# Autodesk Inventor assembly: 3D Printed PCR
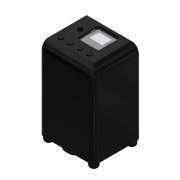
[picture p0: Inventor's stored thumbnail of the model, 180x180]
Saved by Autodesk Inventor 2017 (Build 210142000, 142)
## iProperties
Created: 2017-01-30
Part Number: 3D Printed PCR
Document SubType Name: Assembly
Designer: ge937963
Author: ge937963
## Documents named in this file (8)
- C:\Users\ge937963\Desktop\Inventor View\3D Printed PCR.iam
- C:\Users\ge937963\Desktop\Inventor View\Control Assembly.iam
- C:\Users\ge937963\Desktop\Inventor View\Case.ipt
- C:\Users\ge937963\Desktop\Inventor View\Photodiode Assembly.iam
- C:\Users\ge937963\Desktop\Inventor View\Screw.ipt
- C:\Users\ge937963\Desktop\Inventor View\Battery.ipt
- C:\Users\ge937963\Desktop\Inventor View\Bottom Assembly.iam
- C:\Users\ge937963\Desktop\Inventor View\Cartridge.iam
## Components (11 placed, 7 different names)
1. Control Assembly:1 [sub-assembly] — Flush:1, Flush:2, Mate:1, Mate:5, Mate:6, Mate:7, Mate:8
2. Case:1 — Flush:1, Flush:2, Mate:1, Mate:2, Mate:3, Mate:4, Mate:9, Flush:8, Flush:9, Mate:11, Angle:1
3. Photodiode Assembly:1 [sub-assembly] — Mate:2, Mate:3, Mate:4
4. Screw:1 — Flush:5, Mate:5
5. Screw:2 — Flush:4, Flush:5, Mate:8, Mate:9
6. Screw:3 — Flush:3, Flush:4, Mate:7
7. Screw:4 — Flush:3, Mate:6
8. Battery:1 — Flush:6, Flush:7, Mate:10
9. Battery:2 — Flush:6, Flush:7, Mate:10
10. Bottom Assembly:1 [sub-assembly] — Flush:8, Flush:9, Mate:11, Mate:12
11. Cartridge:1 [sub-assembly] — Mate:12, Angle:1
## Relationships (22: Mate 12, Flush 9, Angle 1)
- Flush:1: Control Assembly:1 ↔ Case:1
- Flush:2: Control Assembly:1 ↔ Case:1
- Mate:1: Control Assembly:1 ↔ Case:1
- Mate:2: Case:1 ↔ Photodiode Assembly:1
- Mate:3: Case:1 ↔ Photodiode Assembly:1
- Mate:4: Case:1 ↔ Photodiode Assembly:1
- Flush:3: Screw:3 ↔ Screw:4
- Flush:4: Screw:2 ↔ Screw:3
- Flush:5: Screw:1 ↔ Screw:2
- Mate:5: Control Assembly:1 ↔ Screw:1
- Mate:6: Control Assembly:1 ↔ Screw:4
- Mate:7: Control Assembly:1 ↔ Screw:3
- Mate:8: Control Assembly:1 ↔ Screw:2
- Mate:9: Case:1 ↔ Screw:2
- Flush:6: Battery:1 ↔ Battery:2
- Flush:7: Battery:1 ↔ Battery:2
- Mate:10 (1 mm): Battery:1 ↔ Battery:2
- Flush:8: Case:1 ↔ Bottom Assembly:1
- Flush:9: Case:1 ↔ Bottom Assembly:1
- Mate:11: Case:1 ↔ Bottom Assembly:1
- Mate:12: Bottom Assembly:1 ↔ Cartridge:1
- Angle:1 (0 deg): Case:1 ↔ Cartridge:1
